# Autodesk Inventor assembly: PFD
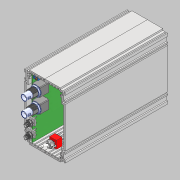
[picture p0: Inventor's stored thumbnail of the model, 180x180]
Saved by Autodesk Inventor 2021.4 (Build 254397000, 397)
## iProperties
Created: 2023-06-23
Part Number: PFD
Document SubType Name: Assembly
Designer: Tilman Preuschoff
Author: Tilman Preuschoff
## Documents named in this file (5)
- C:\Users\Tilman Preuschoff\Documents\GitHub\HMC439_Phase-Frequency_Detector\frontpanel\assembly\PFD.iam
- C:\Users\Tilman Preuschoff\Documents\GitHub\HMC439_Phase-Frequency_Detector\frontpanel\assembly\Fischer HB.ipt
- C:\Users\Tilman Preuschoff\Documents\GitHub\HMC439_Phase-Frequency_Detector\frontpanel\Fischer_TFP.ipt
- C:\Users\Tilman Preuschoff\Documents\GitHub\HMC439_Phase-Frequency_Detector\frontpanel\assembly\phase-frequency_detector.iam
- C:\Users\Tilman Preuschoff\Documents\GitHub\HMC439_Phase-Frequency_Detector\frontpanel\assembly\A203SYCQ04.ipt
## Components (5 placed, 4 different names)
1. Fischer HB:1 — Passend:1, Passend:2, Passend:3, Fluchtend:1, Passend:4, Fluchtend:2, Passend:6, Passend:7, Passend:8, Passend:11
2. Fischer HB:2 — Fluchtend:1, Passend:4, Fluchtend:2, Passend:5
3. Fischer_TFP:1 — Passend:5, Passend:6, Passend:7, Passend:9, Passend:10, Drehbar:1
4. phase-frequency_detector:1 [sub-assembly] — Passend:8, Passend:9, Passend:11
5. A203SYCQ04:1 — Passend:10, Drehbar:1
## Relationships (14: Mate 11, Flush 2, RevoluteJoint 1)
- Passend:1 [Mate]: Fischer HB:1
- Passend:2 [Mate]: Fischer HB:1
- Passend:3 [Mate]: Fischer HB:1
- Fluchtend:1 [Flush]: Fischer HB:1 ↔ Fischer HB:2
- Passend:4 [Mate]: Fischer HB:1 ↔ Fischer HB:2
- Fluchtend:2 [Flush]: Fischer HB:1 ↔ Fischer HB:2
- Passend:5 [Mate]: Fischer HB:2 ↔ Fischer_TFP:1
- Passend:6 [Mate]: Fischer HB:1 ↔ Fischer_TFP:1
- Passend:7 [Mate]: Fischer HB:1 ↔ Fischer_TFP:1
- Passend:8 [Mate]: Fischer HB:1 ↔ phase-frequency_detector:1
- Passend:9 [Mate]: Fischer_TFP:1 ↔ phase-frequency_detector:1
- Passend:10 [Mate]: Fischer_TFP:1 ↔ A203SYCQ04:1
- Drehbar:1 [RevoluteJoint]: Fischer_TFP:1 ↔ A203SYCQ04:1
- Passend:11 [Mate]: Fischer HB:1 ↔ phase-frequency_detector:1
